# Autodesk Inventor assembly: port-cover-2
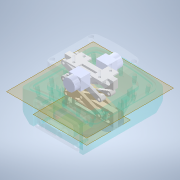
[picture p0: Inventor's stored thumbnail of the model, 180x180]
Saved by Autodesk Inventor 2020 (Build 240168000, 168)
## iProperties
Created: 2019-11-08
Part Number: port-cover-2
Document SubType Name: Assembly
Designer: Hymowitz
Author: Hymowitz
## Documents named in this file (12)
- C:\Users\Hymowitz\Documents\Rocksat2020CAD\port-cover-2.iam
- C:\Users\Hymowitz\Documents\Rocksat2020CAD\MultipurposePort-Released_withSTL\Assembly Multipurpose Port.iam
- C:\Users\Hymowitz\Documents\Rocksat2020CAD\bottom-bracket.ipt
- C:\Users\Hymowitz\Documents\Rocksat2020CAD\bottom slot.ipt
- C:\Users\Hymowitz\Documents\Rocksat2020CAD\screw.ipt
- C:\Users\Hymowitz\Documents\Rocksat2020CAD\3rd party\micro-metal-gearmotor-1000-backshaft.ipt
- C:\Users\Hymowitz\Documents\Rocksat2020CAD\port-cover-2\Design Accelerator\Spur Gears1.iam
- C:\Users\Hymowitz\Documents\Rocksat2020CAD\shuttle.ipt
- C:\Users\Hymowitz\Documents\Rocksat2020CAD\s_arm.ipt
- C:\Users\Hymowitz\Documents\Rocksat2020CAD\cover-holder2.ipt
- C:\Users\Hymowitz\Documents\Rocksat2020CAD\MultipurposePort-Released_withSTL\ME112673.ipt
- C:\Users\Hymowitz\Documents\Rocksat2020CAD\camera.ipt
## Components (19 placed, 11 different names)
1. Assembly Multipurpose Port:1 [sub-assembly] — Flush:1, Flush:2, Mate:1, Mate:8, Mate:9, Mate:38, Mate:39, Flush:8
2. bottom-bracket:1 — Flush:1, Flush:2, Flush:3, Flush:4, Angle:2, Angle:1
3. bottom slot:1 — Flush:3, Mate:2, Mate:3, Mate:4, Flush:5, Mate:8, Mate:9, Mate:14, Mate:15, Mate:16, Mate:17, Flush:7
4. screw:1 — Mate:2, Mate:3, Mate:10, Mate:13
5. micro-metal-gearmotor-1000-backshaft:1 — Flush:4, Mate:4, Flush:5, Mate:11, Mate:12
6. Spur Gears:1 [sub-assembly] — Mate:10, Mate:11, Mate:12
7. shuttle:1 — Mate:13, Angle:1, Mate:22
8. s_arm:1 — Mate:16, Mate:17, Mate:18, Mate:20, Mate:31
9. s_arm:2 — Mate:14, Mate:15, Mate:18, Mate:21, Mate:24, Mate:32
10. s_arm:3 — Mate:21, Mate:22, Mate:23, Mate:24, Mate:33, Mate:34, Mate:40
11. s_arm:4 — Mate:20, Mate:23, Mate:35
12. s_arm:5 — Mate:35
13. s_arm:6 — Mate:33, Mate:34
14. s_arm:7 — Mate:32, Mate:40
15. s_arm:8 — Mate:31, Mate:36
16. cover-holder2:1 — Flush:7, Mate:36, Angle:2, Mate:37
17. ME112673:1 — Mate:37, Mate:38, Mate:39, Mate:41, Flush:9, Flush:10, Flush:11, Mate:42, Flush:12
18. camera:1 — Mate:41, Flush:9, Flush:10
19. camera:2 — Flush:11, Mate:42, Flush:12
## Relationships (52: Mate 39, Flush 11, Angle 2)
- Flush:1: Assembly Multipurpose Port:1 ↔ bottom-bracket:1
- Flush:2: Assembly Multipurpose Port:1 ↔ bottom-bracket:1
- Mate:1: Assembly Multipurpose Port:1
- Flush:3: bottom-bracket:1 ↔ bottom slot:1
- Mate:2: bottom slot:1 ↔ screw:1
- Mate:3: bottom slot:1 ↔ screw:1
- Flush:4 (1 mm): bottom-bracket:1 ↔ micro-metal-gearmotor-1000-backshaft:1
- Mate:4: bottom slot:1 ↔ micro-metal-gearmotor-1000-backshaft:1
- Flush:5: bottom slot:1 ↔ micro-metal-gearmotor-1000-backshaft:1
- Mate:8 (30.48 mm): Assembly Multipurpose Port:1 ↔ bottom slot:1
- Mate:9: Assembly Multipurpose Port:1 ↔ bottom slot:1
- Mate:10: screw:1 ↔ Spur Gears:1
- Mate:11: micro-metal-gearmotor-1000-backshaft:1 ↔ Spur Gears:1
- Mate:12: micro-metal-gearmotor-1000-backshaft:1 ↔ Spur Gears:1
- Mate:13: screw:1 ↔ shuttle:1
- Angle:1 (0 deg): bottom-bracket:1 ↔ shuttle:1
- Mate:14: bottom slot:1 ↔ s_arm:2
- Mate:15: bottom slot:1 ↔ s_arm:2
- Mate:16: bottom slot:1 ↔ s_arm:1
- Mate:17: bottom slot:1 ↔ s_arm:1
- Mate:18: s_arm:1 ↔ s_arm:2
- [Mate]: s_arm:3 ↔ s_arm:4
- Mate:20: s_arm:1 ↔ s_arm:4
- Mate:21: s_arm:2 ↔ s_arm:3
- Mate:22: shuttle:1 ↔ s_arm:3
- Mate:23: s_arm:3 ↔ s_arm:4
- Mate:24: s_arm:2 ↔ s_arm:3
- [Mate]: s_arm:5 ↔ s_arm:6
- [Mate]: s_arm:7 ↔ s_arm:8
- [Mate]: s_arm:5 ↔ s_arm:8
- [Mate]: s_arm:6 ↔ s_arm:7
- [Mate]: s_arm:7 ↔ s_arm:8
- [Mate]: s_arm:6 ↔ s_arm:7
- Mate:31: s_arm:1 ↔ s_arm:8
- Mate:32: s_arm:2 ↔ s_arm:7
- Mate:33: s_arm:3 ↔ s_arm:6
- Mate:34: s_arm:3 ↔ s_arm:6
- Mate:35: s_arm:4 ↔ s_arm:5
- Flush:7: bottom slot:1 ↔ cover-holder2:1
- Mate:36: s_arm:8 ↔ cover-holder2:1
- Angle:2 (0 deg): bottom-bracket:1 ↔ cover-holder2:1
- Mate:37 (-2.032 mm): cover-holder2:1 ↔ ME112673:1
- Mate:38: Assembly Multipurpose Port:1 ↔ ME112673:1
- Mate:39: Assembly Multipurpose Port:1 ↔ ME112673:1
- Mate:40: s_arm:3 ↔ s_arm:7
- Flush:8: Assembly Multipurpose Port:1
- Mate:41: ME112673:1 ↔ camera:1
- Flush:9 (-0.1 mm): ME112673:1 ↔ camera:1
- Flush:10 (24.003 mm): ME112673:1 ↔ camera:1
- Flush:11 (0.2 mm): ME112673:1 ↔ camera:2
- Mate:42 (-3.175 mm): ME112673:1 ↔ camera:2
- Flush:12 (24.003 mm): ME112673:1 ↔ camera:2
## Named parameters: d26_d25 = 0 mm, d42_d25 = 0 mm, d43_d26_d25 = 0 mm, d44_d27 = 0 mm, d45_d28 = 0 mm, d46_d30 = 0 mm, d47_d31 = 0 mm
